# Autodesk Inventor assembly: Base-Rotation
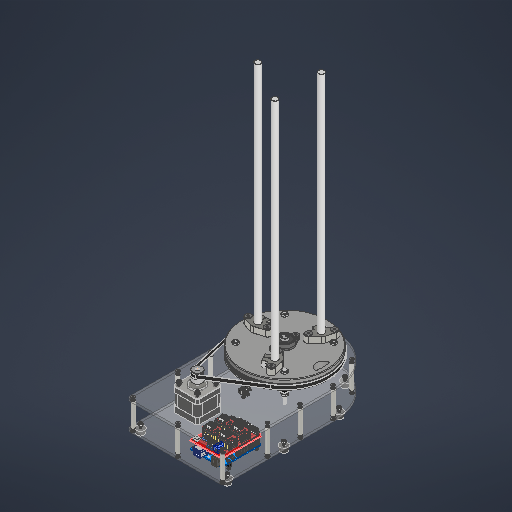
[picture p0: Inventor's stored thumbnail of the model, 512x512]
Saved by Autodesk Inventor 2025.2 (Build 292293000, 293)
## iProperties
Created: 2025-04-10
Part Number: Base-Rotation
Document SubType Name: Assembly
Designer: Tiago
Author: Tiago
## Documents named in this file (30)
- C:\Users\Tiago\Documents\Inventor\Exp. Braço v1\Base-Rotation.iam
- C:\Users\Tiago\Documents\Inventor\Exp. Braço v1\NEMA17 42-38.ipt
- C:\Users\Tiago\Documents\Inventor\Exp. Braço v1\Plataforma_giratoria_4p.iam
- C:\Users\Tiago\Documents\Inventor\Exp. Braço v1\Linear_Shaft_Support_SHF10.ipt
- C:\Users\Tiago\Documents\Inventor\Exp. Braço v1\rodshaft_10x400.ipt
- C:\Users\Tiago\Documents\Inventor\Exp. Braço v1\Base_solida.ipt
- C:\Users\Tiago\Documents\Inventor\Exp. Braço v1\Arduino_CNC_Assembly.iam
- C:\Users\Tiago\Documents\Inventor\Exp. Braço v1\Base_solida_Down.ipt
- C:\Users\Tiago\Documents\Inventor\Exp. Braço v1\Amortecedor_Borracha.ipt
- C:\Users\Tiago\Documents\Inventor\Exp. Braço v1\Espaçador_m3_L3.5.ipt
- C:\Users\Tiago\Documents\Inventor\Exp. Braço v1\espaçador_M3_L40.ipt
- C:\Users\Tiago\Documents\Inventor\Exp. Braço v1\GT2Pulley_z20.ipt
- C:\Users\Tiago\Documents\Inventor\Exp. Braço v1\Base-Rotation\Design Accelerator\Synchronous Belts Transmission3.iam
- C:\Users\Tiago\Documents\Inventor\Exp. Braço v1\Limit_Switch_L1.ipt
- C:\Users\Tiago\Documents\Inventor\Exp. Braço v1\Anilha_M3.ipt
- C:\Users\Tiago\Documents\Inventor\Exp. Braço v1\M3 x0.5 ALT (...).ipt
- C:\Users\Tiago\Documents\Inventor\Exp. Braço v1\Porca_sextavada(4M).ipt
- C:\Users\Tiago\Documents\Inventor\Exp. Braço v1\KFL08 - Mancal Flange oval Ø8.ipt
- C:\Users\Tiago\Documents\Inventor\Exp. Braço v1\M3 x8L_hexagonal_BigHEAD.ipt
- C:\Users\Tiago\Documents\Inventor\Exp. Braço v1\M3 x5L_hexagonal.ipt
- C:\Users\Tiago\Documents\Inventor\Exp. Braço v1\M4x22L_Hex.ipt
- C:\Users\Tiago\Documents\Inventor\Exp. Braço v1\M5 x12L_Hex_C.ipt
- M5 x12L_Hex_C.ipt
- C:\Users\Tiago\Documents\Inventor\Exp. Braço v1\M5x16L_Hex.ipt
- C:\Users\Tiago\Documents\Inventor\Exp. Braço v1\Porca_sextavada(3M).ipt
- C:\Users\Tiago\Documents\Inventor\Exp. Braço v1\M2x12L_Hex.ipt
- M2x12L_Hex.ipt
- C:\Users\Tiago\Documents\Inventor\Exp. Braço v1\Porca_sextavada(M2).ipt
- C:\Users\Tiago\Documents\Inventor\Exp. Braço v1\M5_nylonLock_Nut.ipt
- C:\Users\Tiago\Documents\Inventor\Exp. Braço v1\PoliaDentada220dentes.ipt
## Components (135 placed, 27 different names)
1. NEMA17 42-38:1 — Mate:85, Mate:86, Flush:4, Mate:87, Flush:8
2. Plataforma_giratoria_4p:1 [sub-assembly] — Mate:27, Mate:28, Mate:29, Insert:117, Insert:118, Insert:119, Insert:120, Insert:121, Insert:122, Insert:123, Insert:124, Mate:168, Mate:169, Mate:170, Angle:1
3. Linear_Shaft_Support_SHF10:1 — Mate:20, Insert:129, Insert:138, Insert:139, Mate:173, Mate:174
4. Linear_Shaft_Support_SHF10:2 — Mate:21, Mate:133, Insert:131, Insert:134, Insert:135, Mate:177, Mate:178
5. Linear_Shaft_Support_SHF10:3 — Mate:22, Insert:130, Insert:136, Insert:137, Mate:179, Mate:182
6. rodshaft_10x400:1 — Mate:22, Mate:180, Mate:181
7. rodshaft_10x400:2 — Mate:21, Mate:133, Mate:175, Mate:176
8. rodshaft_10x400:3 — Mate:20, Mate:171, Mate:172
9. Base_solida:1 — Mate:27, Mate:28, Mate:29, Mate:31, Flush:1, Flush:2, Mate:85, Mate:87, Mate:97, Mate:98, Flush:8, Mate:102, Mate:107, Mate:111, Mate:112, Mate:113, Mate:115, Mate:117, Mate:119, Mate:121, Mate:166, Mate:167, Insert:150, Insert:151, Insert:162, Insert:163, Insert:164, Insert:165, Insert:166, Insert:167, Insert:168, Insert:169, Insert:170, Insert:171, Insert:172, Insert:173
10. Arduino_CNC_Assembly:1 [sub-assembly] — Mate:32, Mate:33, Mate:34, Mate:35, Mate:36, Insert:111, Insert:114, Insert:115, Insert:116
11. Base_solida_Down:1 — Mate:31, Flush:1, Flush:2, Mate:32, Mate:33, Mate:34, Mate:35, Mate:36, Mate:37, Mate:38, Mate:39, Mate:40, Mate:41, Mate:42, Mate:43, Mate:44, Mate:54, Mate:55, Mate:56, Mate:57, Mate:58, Mate:59, Mate:61, Mate:62, Mate:63, Mate:64, Mate:65, Mate:66, Mate:67, Mate:68, Mate:69, Mate:70, Mate:71, Mate:72, Mate:73, Mate:74, Mate:75, Mate:76, Mate:77, Mate:78, Mate:79, Mate:80, Mate:81, Mate:82, Mate:83, Mate:84, Flush:7, Mate:153, Mate:154, Insert:95, Insert:96, Mate:155, Mate:156, Mate:157, Mate:158, Mate:159, Mate:160, Mate:161, Mate:162, Insert:112, Insert:113, Insert:140, Insert:141, Insert:142, Insert:143, Insert:144, Insert:145, Insert:146, Insert:147, Insert:152, Insert:153, Insert:154, Insert:155, Insert:156, Insert:157, Insert:158, Insert:159, Insert:160, Insert:161, Insert:175, Insert:176
12. Amortecedor_Borracha:1 — Mate:57, Mate:159, Insert:102
13. Amortecedor_Borracha:2 — Mate:58, Mate:160, Insert:100
14. Amortecedor_Borracha:3 — Mate:59, Mate:161, Insert:99
15. Amortecedor_Borracha:4 — Mate:56, Mate:158, Insert:101
16. Amortecedor_Borracha:5 — Mate:153, Mate:162, Insert:98
17. Amortecedor_Borracha:6 — Mate:54, Mate:156, Mate:164
18. Amortecedor_Borracha:7 — Mate:154, Mate:155, Insert:97
19. Amortecedor_Borracha:8 — Mate:55, Mate:157, Mate:163
20. Espaçador_m3_L3.5:1 — Mate:37, Mate:41
21. Espaçador_m3_L3.5:2 — Mate:38, Mate:44
22. Espaçador_m3_L3.5:3 — Mate:40, Mate:42
23. Espaçador_m3_L3.5:4 — Mate:39, Mate:43
24. espaçador_M3_L40:1 — Mate:61, Mate:73
25. espaçador_M3_L40:2 — Mate:62, Mate:75
26. espaçador_M3_L40:3 — Mate:63, Mate:76
27. espaçador_M3_L40:4 — Mate:64, Mate:77
28. espaçador_M3_L40:5 — Mate:65, Mate:78
29. espaçador_M3_L40:6 — Mate:66, Mate:79
30. espaçador_M3_L40:7 — Mate:67, Mate:74
31. espaçador_M3_L40:8 — Mate:68, Mate:84
32. espaçador_M3_L40:9 — Mate:69, Mate:83
33. espaçador_M3_L40:10 — Mate:70, Mate:82
34. espaçador_M3_L40:11 — Mate:71, Mate:81
35. espaçador_M3_L40:12 — Mate:72, Mate:80
36. GT2Pulley_z20:1 — Mate:86, Flush:4, Mate:96, Flush:6
37. Synchronous Belts Transmission:1 [sub-assembly] — Mate:96, Flush:6
38. Limit_Switch_L1:1 — Mate:102, Mate:166, Mate:167, Insert:148, Insert:149
39. M3 x0.5 ALT (...):1 — Insert:162
40. M3 x0.5 ALT (...):2 — Insert:164
41. M3 x0.5 ALT (...):3 — Insert:165
42. M3 x0.5 ALT (...):4 — Insert:166
43. M3 x0.5 ALT (...):5 — Insert:167
44. M3 x0.5 ALT (...):6 — Insert:168
45. M3 x0.5 ALT (...):7 — Insert:169
46. M3 x0.5 ALT (...):8 — Insert:173
47. M3 x0.5 ALT (...):9 — Insert:172
48. M3 x0.5 ALT (...):10 — Insert:171
49. M3 x0.5 ALT (...):11 — Insert:170
50. M3 x0.5 ALT (...):12 — Insert:163
51. M3 x0.5 ALT (...):13 — Insert:156
52. M3 x0.5 ALT (...):14 — Insert:155
53. M3 x0.5 ALT (...):15 — Insert:154
54. M3 x0.5 ALT (...):16 — Insert:153
55. M3 x0.5 ALT (...):17 — Insert:152
56. M3 x0.5 ALT (...):18 — Insert:96
57. M3 x0.5 ALT (...):19 — Insert:161
58. M3 x0.5 ALT (...):20 — Insert:159
59. M3 x0.5 ALT (...):21 — Insert:160
60. M3 x0.5 ALT (...):22 — Insert:158
61. M3 x0.5 ALT (...):23 — Insert:157
62. M3 x0.5 ALT (...):24 — Insert:95
63. Anilha_M3:25 — Mate:107, Insert:106
64. Anilha_M3:26 — Mate:113, Insert:105
65. Anilha_M3:27 — Mate:112, Insert:104
66. Anilha_M3:28 — Mate:111, Insert:103
67. Porca_sextavada(4M):1 — Mate:115
68. Porca_sextavada(4M):2 — Mate:117
69. Porca_sextavada(4M):3 — Mate:119
70. Porca_sextavada(4M):4 — Mate:121
71. Porca_sextavada(4M):5
72. Porca_sextavada(4M):6
73. Porca_sextavada(4M):7
74. Porca_sextavada(4M):8 — Insert:177
75. KFL08 - Mancal Flange oval Ø8:1 — Insert:133, Insert:174
76. M3 x0.5 ALT (...):29 — Insert:98
77. M3 x0.5 ALT (...):30 — Insert:97
78. M3 x0.5 ALT (...):31 — Insert:99
79. M3 x0.5 ALT (...):32 — Insert:100
80. M3 x0.5 ALT (...):33 — Insert:101
81. M3 x0.5 ALT (...):34 — Insert:102
82. M3 x0.5 ALT (...):35 — Mate:163
83. M3 x0.5 ALT (...):36 — Mate:164
84. M3 x8L_hexagonal_BigHEAD:1 — Insert:103
85. M3 x8L_hexagonal_BigHEAD:2 — Insert:104
86. M3 x8L_hexagonal_BigHEAD:3 — Insert:105
87. M3 x8L_hexagonal_BigHEAD:4 — Insert:106
88. M3 x5L_hexagonal:1 — Insert:175
89. M3 x5L_hexagonal:2 — Insert:176
90. M3 x5L_hexagonal:3 — Insert:112
91. M3 x5L_hexagonal:4 — Insert:113
92. M3 x5L_hexagonal:5 — Insert:111
93. M3 x5L_hexagonal:6 — Insert:114
94. M3 x5L_hexagonal:7 — Insert:115
95. M3 x5L_hexagonal:8 — Insert:116
96. M4x22L_Hex:1 — Insert:117
97. M4x22L_Hex:2 — Insert:118
98. M4x22L_Hex:3 — Insert:120
99. M4x22L_Hex:4 — Insert:121
100. M4x22L_Hex:5 — Insert:123
101. M4x22L_Hex:6 — Insert:122
102. M4x22L_Hex:7 — Insert:119
103. M4x22L_Hex:8 — Insert:124
104. M5 x12L_Hex_C:1 — Insert:129
105. M5 x12L_Hex_C:2 — Insert:130
106. M5 x12L_Hex_C:3 — Insert:131
107. M5x16L_Hex:1 — Insert:174
108. M5x16L_Hex:2 — Insert:133
109. M5x16L_Hex:3 — Insert:137
110. M5x16L_Hex:4 — Insert:135
111. M5x16L_Hex:5 — Insert:136
112. M5x16L_Hex:6 — Insert:139
113. M5x16L_Hex:7 — Insert:138
114. M5x16L_Hex:8 — Insert:134
115. Porca_sextavada(3M):1 — Insert:140
116. Porca_sextavada(3M):2 — Insert:142
117. Porca_sextavada(3M):3 — Insert:141
118. Porca_sextavada(3M):4 — Insert:143
119. Porca_sextavada(3M):5 — Insert:144
120. Porca_sextavada(3M):6 — Insert:147
121. Porca_sextavada(3M):7 — Insert:146
122. Porca_sextavada(3M):8 — Insert:145
123. M2x12L_Hex:1 — Insert:149
124. M2x12L_Hex:2 — Insert:148
125. Porca_sextavada(M2):1 — Insert:151
126. Porca_sextavada(M2):2 — Insert:150
127. M5_nylonLock_Nut:1 — Insert:180
128. M5_nylonLock_Nut:2 — Insert:178
129. M5_nylonLock_Nut:3 — Insert:179
130. M5_nylonLock_Nut:4
131. M5_nylonLock_Nut:5
132. M5_nylonLock_Nut:6
133. M5_nylonLock_Nut:7
134. M5_nylonLock_Nut:8
135. PoliaDentada220dentes:1 — Mate:168, Mate:169, Mate:170, Angle:1, Insert:177, Mate:171, Mate:172, Mate:173, Mate:174, Insert:178, Insert:179, Insert:180, Mate:175, Mate:176, Mate:177, Mate:178, Mate:179, Mate:180, Mate:181, Mate:182
## Relationships (179: Mate 95, Insert 77, Flush 6, Angle 1)
- Mate:20: Linear_Shaft_Support_SHF10:1 ↔ rodshaft_10x400:3
- Mate:21: Linear_Shaft_Support_SHF10:2 ↔ rodshaft_10x400:2
- Mate:22: Linear_Shaft_Support_SHF10:3 ↔ rodshaft_10x400:1
- Mate:27: Plataforma_giratoria_4p:1 ↔ Base_solida:1
- Mate:28: Plataforma_giratoria_4p:1 ↔ Base_solida:1
- Mate:29: Plataforma_giratoria_4p:1 ↔ Base_solida:1
- Mate:31 (40 mm): Base_solida:1 ↔ Base_solida_Down:1
- Flush:1: Base_solida:1 ↔ Base_solida_Down:1
- Flush:2: Base_solida:1 ↔ Base_solida_Down:1
- Mate:32 (5 mm): Arduino_CNC_Assembly:1 ↔ Base_solida_Down:1
- Mate:33: Arduino_CNC_Assembly:1 ↔ Base_solida_Down:1
- Mate:34: Arduino_CNC_Assembly:1 ↔ Base_solida_Down:1
- Mate:35: Arduino_CNC_Assembly:1 ↔ Base_solida_Down:1
- Mate:36: Arduino_CNC_Assembly:1 ↔ Base_solida_Down:1
- Mate:37: Base_solida_Down:1 ↔ Espaçador_m3_L3.5:1
- Mate:38: Base_solida_Down:1 ↔ Espaçador_m3_L3.5:2
- Mate:39: Base_solida_Down:1 ↔ Espaçador_m3_L3.5:4
- Mate:40: Base_solida_Down:1 ↔ Espaçador_m3_L3.5:3
- Mate:41: Base_solida_Down:1 ↔ Espaçador_m3_L3.5:1
- Mate:42: Base_solida_Down:1 ↔ Espaçador_m3_L3.5:3
- Mate:43: Base_solida_Down:1 ↔ Espaçador_m3_L3.5:4
- Mate:44: Base_solida_Down:1 ↔ Espaçador_m3_L3.5:2
- Mate:54: Base_solida_Down:1 ↔ Amortecedor_Borracha:6
- Mate:55: Base_solida_Down:1 ↔ Amortecedor_Borracha:8
- Mate:56: Base_solida_Down:1 ↔ Amortecedor_Borracha:4
- Mate:57: Base_solida_Down:1 ↔ Amortecedor_Borracha:1
- Mate:58: Base_solida_Down:1 ↔ Amortecedor_Borracha:2
- Mate:59: Base_solida_Down:1 ↔ Amortecedor_Borracha:3
- Mate:61: Base_solida_Down:1 ↔ espaçador_M3_L40:1
- Mate:62: Base_solida_Down:1 ↔ espaçador_M3_L40:2
- Mate:63: Base_solida_Down:1 ↔ espaçador_M3_L40:3
- Mate:64: Base_solida_Down:1 ↔ espaçador_M3_L40:4
- Mate:65: Base_solida_Down:1 ↔ espaçador_M3_L40:5
- Mate:66: Base_solida_Down:1 ↔ espaçador_M3_L40:6
- Mate:67: Base_solida_Down:1 ↔ espaçador_M3_L40:7
- Mate:68: Base_solida_Down:1 ↔ espaçador_M3_L40:8
- Mate:69: Base_solida_Down:1 ↔ espaçador_M3_L40:9
- Mate:70: Base_solida_Down:1 ↔ espaçador_M3_L40:10
- Mate:71: Base_solida_Down:1 ↔ espaçador_M3_L40:11
- Mate:72: Base_solida_Down:1 ↔ espaçador_M3_L40:12
- Mate:73: Base_solida_Down:1 ↔ espaçador_M3_L40:1
- Mate:74: Base_solida_Down:1 ↔ espaçador_M3_L40:7
- Mate:75: Base_solida_Down:1 ↔ espaçador_M3_L40:2
- Mate:76: Base_solida_Down:1 ↔ espaçador_M3_L40:3
- Mate:77: Base_solida_Down:1 ↔ espaçador_M3_L40:4
- Mate:78: Base_solida_Down:1 ↔ espaçador_M3_L40:5
- Mate:79: Base_solida_Down:1 ↔ espaçador_M3_L40:6
- Mate:80: Base_solida_Down:1 ↔ espaçador_M3_L40:12
- Mate:81: Base_solida_Down:1 ↔ espaçador_M3_L40:11
- Mate:82: Base_solida_Down:1 ↔ espaçador_M3_L40:10
- Mate:83: Base_solida_Down:1 ↔ espaçador_M3_L40:9
- Mate:84: Base_solida_Down:1 ↔ espaçador_M3_L40:8
- Mate:85: NEMA17 42-38:1 ↔ Base_solida:1
- Mate:86: NEMA17 42-38:1 ↔ GT2Pulley_z20:1
- Flush:4 (-0.8 mm): NEMA17 42-38:1 ↔ GT2Pulley_z20:1
- Mate:87: NEMA17 42-38:1 ↔ Base_solida:1
- Mate:96: GT2Pulley_z20:1 ↔ Synchronous Belts Transmission:1
- Flush:6 (2 mm): GT2Pulley_z20:1 ↔ Synchronous Belts Transmission:1
- Flush:7: Base_solida_Down:1
- Mate:97: Base_solida:1
- Mate:98: Base_solida:1
- Flush:8 (59.286 mm): NEMA17 42-38:1 ↔ Base_solida:1
- Mate:102: Base_solida:1 ↔ Limit_Switch_L1:1
- Mate:107: Base_solida:1 ↔ Anilha_M3:25
- Mate:111: Base_solida:1 ↔ Anilha_M3:28
- Mate:112: Base_solida:1 ↔ Anilha_M3:27
- Mate:113: Base_solida:1 ↔ Anilha_M3:26
- Mate:115: Base_solida:1 ↔ Porca_sextavada(4M):1
- Mate:117: Base_solida:1 ↔ Porca_sextavada(4M):2
- Mate:119: Base_solida:1 ↔ Porca_sextavada(4M):3
- Mate:121: Base_solida:1 ↔ Porca_sextavada(4M):4
- Mate:133: Linear_Shaft_Support_SHF10:2 ↔ rodshaft_10x400:2
- Mate:153: Base_solida_Down:1 ↔ Amortecedor_Borracha:5
- Mate:154: Base_solida_Down:1 ↔ Amortecedor_Borracha:7
- Insert:95: Base_solida_Down:1 ↔ M3 x0.5 ALT (...):24
- Insert:96: Base_solida_Down:1 ↔ M3 x0.5 ALT (...):18
- Mate:155: Base_solida_Down:1 ↔ Amortecedor_Borracha:7
- Insert:97: Amortecedor_Borracha:7 ↔ M3 x0.5 ALT (...):30
- Mate:156: Base_solida_Down:1 ↔ Amortecedor_Borracha:6
- Mate:157: Base_solida_Down:1 ↔ Amortecedor_Borracha:8
- Mate:158: Base_solida_Down:1 ↔ Amortecedor_Borracha:4
- Mate:159: Base_solida_Down:1 ↔ Amortecedor_Borracha:1
- Mate:160: Base_solida_Down:1 ↔ Amortecedor_Borracha:2
- Mate:161: Base_solida_Down:1 ↔ Amortecedor_Borracha:3
- Mate:162: Base_solida_Down:1 ↔ Amortecedor_Borracha:5
- Insert:98: Amortecedor_Borracha:5 ↔ M3 x0.5 ALT (...):29
- Insert:99: Amortecedor_Borracha:3 ↔ M3 x0.5 ALT (...):31
- Insert:100: Amortecedor_Borracha:2 ↔ M3 x0.5 ALT (...):32
- Insert:101: Amortecedor_Borracha:4 ↔ M3 x0.5 ALT (...):33
- Insert:102: Amortecedor_Borracha:1 ↔ M3 x0.5 ALT (...):34
- Mate:163: Amortecedor_Borracha:8 ↔ M3 x0.5 ALT (...):35
- Mate:164: Amortecedor_Borracha:6 ↔ M3 x0.5 ALT (...):36
- Insert:103: Anilha_M3:28 ↔ M3 x8L_hexagonal_BigHEAD:1
- Insert:104: Anilha_M3:27 ↔ M3 x8L_hexagonal_BigHEAD:2
- Insert:105: Anilha_M3:26 ↔ M3 x8L_hexagonal_BigHEAD:3
- Insert:106: Anilha_M3:25 ↔ M3 x8L_hexagonal_BigHEAD:4
- Insert:111: Arduino_CNC_Assembly:1 ↔ M3 x5L_hexagonal:5
- Insert:112: Base_solida_Down:1 ↔ M3 x5L_hexagonal:3
- Insert:113: Base_solida_Down:1 ↔ M3 x5L_hexagonal:4
- Insert:114: Arduino_CNC_Assembly:1 ↔ M3 x5L_hexagonal:6
- Insert:115: Arduino_CNC_Assembly:1 ↔ M3 x5L_hexagonal:7
- Insert:116: Arduino_CNC_Assembly:1 ↔ M3 x5L_hexagonal:8
- Insert:117: Plataforma_giratoria_4p:1 ↔ M4x22L_Hex:1
- Insert:118: Plataforma_giratoria_4p:1 ↔ M4x22L_Hex:2
- Insert:119: Plataforma_giratoria_4p:1 ↔ M4x22L_Hex:7
- Insert:120: Plataforma_giratoria_4p:1 ↔ M4x22L_Hex:3
- Insert:121: Plataforma_giratoria_4p:1 ↔ M4x22L_Hex:4
- Insert:122: Plataforma_giratoria_4p:1 ↔ M4x22L_Hex:6
- Insert:123: Plataforma_giratoria_4p:1 ↔ M4x22L_Hex:5
- Insert:124: Plataforma_giratoria_4p:1 ↔ M4x22L_Hex:8
- Insert:129: Linear_Shaft_Support_SHF10:1 ↔ M5 x12L_Hex_C:1
- Insert:130: Linear_Shaft_Support_SHF10:3 ↔ M5 x12L_Hex_C:2
- Insert:131: Linear_Shaft_Support_SHF10:2 ↔ M5 x12L_Hex_C:3
- Insert:133: KFL08 - Mancal Flange oval Ø8:1 ↔ M5x16L_Hex:2
- Insert:134: Linear_Shaft_Support_SHF10:2 ↔ M5x16L_Hex:8
- Insert:135: Linear_Shaft_Support_SHF10:2 ↔ M5x16L_Hex:4
- Insert:136: Linear_Shaft_Support_SHF10:3 ↔ M5x16L_Hex:5
- Insert:137: Linear_Shaft_Support_SHF10:3 ↔ M5x16L_Hex:3
- Insert:138: Linear_Shaft_Support_SHF10:1 ↔ M5x16L_Hex:7
- Insert:139: Linear_Shaft_Support_SHF10:1 ↔ M5x16L_Hex:6
- Insert:140: Base_solida_Down:1 ↔ Porca_sextavada(3M):1
- Insert:141: Base_solida_Down:1 ↔ Porca_sextavada(3M):3
- Insert:142: Base_solida_Down:1 ↔ Porca_sextavada(3M):2
- Insert:143: Base_solida_Down:1 ↔ Porca_sextavada(3M):4
- Insert:144: Base_solida_Down:1 ↔ Porca_sextavada(3M):5
- Insert:145: Base_solida_Down:1 ↔ Porca_sextavada(3M):8
- Insert:146: Base_solida_Down:1 ↔ Porca_sextavada(3M):7
- Insert:147: Base_solida_Down:1 ↔ Porca_sextavada(3M):6
- Mate:166: Base_solida:1 ↔ Limit_Switch_L1:1
- Mate:167: Base_solida:1 ↔ Limit_Switch_L1:1
- Insert:148: Limit_Switch_L1:1 ↔ M2x12L_Hex:2
- Insert:149: Limit_Switch_L1:1 ↔ M2x12L_Hex:1
- Insert:150: Base_solida:1 ↔ Porca_sextavada(M2):2
- Insert:151: Base_solida:1 ↔ Porca_sextavada(M2):1
- Insert:152: Base_solida_Down:1 ↔ M3 x0.5 ALT (...):17
- Insert:153: Base_solida_Down:1 ↔ M3 x0.5 ALT (...):16
- Insert:154: Base_solida_Down:1 ↔ M3 x0.5 ALT (...):15
- Insert:155: Base_solida_Down:1 ↔ M3 x0.5 ALT (...):14
- Insert:156: Base_solida_Down:1 ↔ M3 x0.5 ALT (...):13
- Insert:157: Base_solida_Down:1 ↔ M3 x0.5 ALT (...):23
- Insert:158: Base_solida_Down:1 ↔ M3 x0.5 ALT (...):22
- Insert:159: Base_solida_Down:1 ↔ M3 x0.5 ALT (...):20
- Insert:160: Base_solida_Down:1 ↔ M3 x0.5 ALT (...):21
- Insert:161: Base_solida_Down:1 ↔ M3 x0.5 ALT (...):19
- Insert:162: Base_solida:1 ↔ M3 x0.5 ALT (...):1
- Insert:163: Base_solida:1 ↔ M3 x0.5 ALT (...):12
- Insert:164: Base_solida:1 ↔ M3 x0.5 ALT (...):2
- Insert:165: Base_solida:1 ↔ M3 x0.5 ALT (...):3
- Insert:166: Base_solida:1 ↔ M3 x0.5 ALT (...):4
- Insert:167: Base_solida:1 ↔ M3 x0.5 ALT (...):5
- Insert:168: Base_solida:1 ↔ M3 x0.5 ALT (...):6
- Insert:169: Base_solida:1 ↔ M3 x0.5 ALT (...):7
- Insert:170: Base_solida:1 ↔ M3 x0.5 ALT (...):11
- Insert:171: Base_solida:1 ↔ M3 x0.5 ALT (...):10
- Insert:172: Base_solida:1 ↔ M3 x0.5 ALT (...):9
- Insert:173: Base_solida:1 ↔ M3 x0.5 ALT (...):8
- Insert:174: KFL08 - Mancal Flange oval Ø8:1 ↔ M5x16L_Hex:1
- Insert:175: Base_solida_Down:1 ↔ M3 x5L_hexagonal:1
- Insert:176: Base_solida_Down:1 ↔ M3 x5L_hexagonal:2
- Mate:168: Plataforma_giratoria_4p:1 ↔ PoliaDentada220dentes:1
- Mate:169: Plataforma_giratoria_4p:1 ↔ PoliaDentada220dentes:1
- Mate:170: Plataforma_giratoria_4p:1 ↔ PoliaDentada220dentes:1
- Angle:1 (0 deg): Plataforma_giratoria_4p:1 ↔ PoliaDentada220dentes:1
- Insert:177: Porca_sextavada(4M):8 ↔ PoliaDentada220dentes:1
- Mate:171: rodshaft_10x400:3 ↔ PoliaDentada220dentes:1
- Mate:172: rodshaft_10x400:3 ↔ PoliaDentada220dentes:1
- Mate:173: Linear_Shaft_Support_SHF10:1 ↔ PoliaDentada220dentes:1
- Mate:174: Linear_Shaft_Support_SHF10:1 ↔ PoliaDentada220dentes:1
- Insert:178: M5_nylonLock_Nut:2 ↔ PoliaDentada220dentes:1
- Insert:179: M5_nylonLock_Nut:3 ↔ PoliaDentada220dentes:1
- Insert:180: M5_nylonLock_Nut:1 ↔ PoliaDentada220dentes:1
- Mate:175: rodshaft_10x400:2 ↔ PoliaDentada220dentes:1
- Mate:176: rodshaft_10x400:2 ↔ PoliaDentada220dentes:1
- Mate:177: Linear_Shaft_Support_SHF10:2 ↔ PoliaDentada220dentes:1
- Mate:178: Linear_Shaft_Support_SHF10:2 ↔ PoliaDentada220dentes:1
- Mate:179: Linear_Shaft_Support_SHF10:3 ↔ PoliaDentada220dentes:1
- Mate:180: rodshaft_10x400:1 ↔ PoliaDentada220dentes:1
- Mate:181: rodshaft_10x400:1 ↔ PoliaDentada220dentes:1
- Mate:182: Linear_Shaft_Support_SHF10:3 ↔ PoliaDentada220dentes:1
